# Autodesk Inventor assembly: Final Assembly
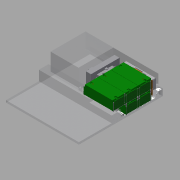
[picture p0: Inventor's stored thumbnail of the model, 180x180]
Saved by Autodesk Inventor 2017 (Build 210142000, 142)
## iProperties
Created: 2022-08-16
Part Number: Final Assembly
Document SubType Name: Assembly
Designer: JTS
Author: JTS
## Documents named in this file (18)
- C:\Users\Windermac\Desktop\MASTER Honda Insight G1 IMA Bay\02 Final Assembly (Tray Mated).iam
- C:\Users\Windermac\Desktop\MASTER Honda Insight G1 IMA Bay\LiBCM003 - Battery Tray\47 Ah FoMoCo Aluminum Tray.ipt
- C:\Users\Windermac\Desktop\MASTER Honda Insight G1 IMA Bay\OEM Parts\Junction Board.ipt
- C:\Users\Windermac\Desktop\MASTER Honda Insight G1 IMA Bay\OEM Parts\MCM.ipt
- C:\Users\Windermac\Desktop\MASTER Honda Insight G1 IMA Bay\Battery Modules\47Ah-FoMoCo.ipt
- C:\Users\Windermac\Desktop\MASTER Honda Insight G1 IMA Bay\LiBCM004 - Battery Rail\Bracket - 5th Module 8982K875.ipt
- C:\Users\Windermac\Desktop\MASTER Honda Insight G1 IMA Bay\Nuts & Bolts\Ring Terminal.ipt
- C:\Users\Windermac\Desktop\MASTER Honda Insight G1 IMA Bay\Final Assembly\AIP\Cable and Harness\Final Assembly.Harness2.iam
- C:\Users\Windermac\Desktop\MASTER Honda Insight G1 IMA Bay\LiBCM PCB\LiBCM Safety Cover - RevC.ipt
- C:\Users\Windermac\Desktop\MASTER Honda Insight G1 IMA Bay\LiBCM PCB\PCB.ipt
- C:\Users\Windermac\Desktop\MASTER Honda Insight G1 IMA Bay\OEM Parts\IMA Bay - Battery Enclosure Interface.ipt
- C:\Users\Windermac\Desktop\MASTER Honda Insight G1 IMA Bay\Nuts & Bolts\Battery Bolt.iam
- C:\Users\Windermac\Desktop\MASTER Honda Insight G1 IMA Bay\Nuts & Bolts\Threaded Standoff.ipt
- C:\Users\Windermac\Desktop\MASTER Honda Insight G1 IMA Bay\Nuts & Bolts\Battery Bolt - Split Washer.iam
- C:\Users\Windermac\Desktop\MASTER Honda Insight G1 IMA Bay\Nuts & Bolts\Washer 0.250in 92141A029.ipt
- C:\Users\Windermac\Desktop\MASTER Honda Insight G1 IMA Bay\Nuts & Bolts\Nut - Hex - 0.250in-20 91845A029.ipt
- C:\Users\Windermac\Desktop\MASTER Honda Insight G1 IMA Bay\Nuts & Bolts\Washer - Split - 92146A029.ipt
- C:\Users\Windermac\Desktop\MASTER Honda Insight G1 IMA Bay\Nuts & Bolts\Top Spacer.ipt
## Components (63 placed, 17 different names)
1. IMA Bay - Battery Enclosure Interface:1 — Insert:56, Mate:2, Mate:3, Mate:4
2. Junction Board:1 — Insert:11, Insert:12
3. MCM:1 — Insert:9, Insert:10
4. Harness2 [sub-assembly]
5. Washer 0.250in 92141A029:3 — Insert:124
6. Nut - Hex - 0.250in-20 91845A029:5
7. Top Spacer:1 — Insert:125, Insert:126
8. 47 Ah FoMoCo Aluminum Tray:1 — Insert:9, Insert:10, Insert:11, Insert:12, Insert:56, Mate:2, Insert:97, Insert:98, Insert:99, Insert:100, Insert:101, Insert:102, Insert:103, Insert:104, Insert:105, Insert:106, Insert:107, Insert:108, Insert:124
9. LiBCM Safety Cover - RevC:1 — Insert:55, Mate:1, Mate:3, Flush:1, Mate:4
10. PCB:1 — Insert:55, Mate:1
11. Threaded Standoff:1 — Insert:65
12. Threaded Standoff:2 — Insert:70
13. Threaded Standoff:3 — Insert:71
14. Threaded Standoff:4 — Insert:72, Insert:114
15. Threaded Standoff:5 — Insert:69, Insert:113
16. Threaded Standoff:6 — Insert:68, Insert:110
17. Threaded Standoff:7 — Insert:67
18. Threaded Standoff:8 — Insert:66, Insert:109
19. Battery Bolt:1 [sub-assembly] — Insert:102
20. Battery Bolt:2 [sub-assembly] — Insert:101
21. Battery Bolt:3 [sub-assembly] — Insert:99
22. Battery Bolt:4 [sub-assembly] — Insert:98
23. Battery Bolt:5 [sub-assembly] — Insert:100
24. Battery Bolt:6 [sub-assembly] — Insert:104
25. Battery Bolt:7 [sub-assembly] — Insert:103
26. Battery Bolt:8 [sub-assembly] — Insert:97
27. 47Ah-FoMoCo:1 — Insert:41, Insert:43, Tangent:1, Tangent:7, Insert:65, Insert:66, Insert:71, Insert:72, Insert:107, Insert:108
28. 47Ah-FoMoCo:2 — Insert:42, Insert:44, Tangent:3, Tangent:13, Insert:67, Insert:68, Insert:69, Insert:70, Insert:105, Insert:106
29. Bracket - 5th Module 8982K875:1 — Insert:109, Insert:110, Insert:111, Insert:112, Insert:120, Insert:121, Insert:122
30. Bracket - 5th Module 8982K875:2 — Insert:113, Insert:114, Insert:115, Insert:116, Insert:117, Insert:118, Insert:119
31. Battery Bolt:9 [sub-assembly] — Insert:115
32. Battery Bolt:10 [sub-assembly] — Insert:116
33. Washer 0.250in 92141A029:1 — Insert:91, Insert:112
34. Washer 0.250in 92141A029:2 — Insert:92, Insert:111
35. Nut - Hex - 0.250in-20 91845A029:1 — Insert:91
36. Nut - Hex - 0.250in-20 91845A029:2 — Insert:92
37. Washer - Split - 92146A029:1 — Insert:93, Insert:95
38. Washer - Split - 92146A029:2 — Insert:94, Insert:96
39. Nut - Hex - 0.250in-20 91845A029:3 — Insert:96
40. Nut - Hex - 0.250in-20 91845A029:4 — Insert:95
41. Battery Bolt - Split Washer:1 [sub-assembly] — Insert:77
42. Battery Bolt - Split Washer:2 [sub-assembly] — Insert:78
43. Battery Bolt - Split Washer:3 [sub-assembly] — Insert:79
44. Battery Bolt - Split Washer:4 [sub-assembly] — Insert:80
45. Battery Bolt - Split Washer:5 [sub-assembly] — Insert:84
46. Battery Bolt - Split Washer:6 [sub-assembly] — Insert:83
47. Battery Bolt - Split Washer:7 [sub-assembly] — Insert:82
48. Battery Bolt - Split Washer:8 [sub-assembly] — Insert:81
49. Battery Bolt - Split Washer:9 [sub-assembly] — Insert:126
50. Battery Bolt - Split Washer:10 [sub-assembly] — Insert:85
51. 47Ah-FoMoCo:3 — Insert:37, Insert:40, Tangent:9, Tangent:12, Flush:1, Insert:79, Insert:80, Insert:81, Insert:82, Insert:121, Insert:122
52. 47Ah-FoMoCo:4 — Insert:36, Insert:39, Tangent:14, Tangent:15, Insert:77, Insert:78, Insert:83, Insert:84, Insert:119, Insert:120
53. 47Ah-FoMoCo:5 — Insert:35, Insert:38, Tangent:16, Tangent:17, Insert:85, Insert:93, Insert:94, Insert:117, Insert:118, Insert:125
54. Ring Terminal:1 — Insert:35, Tangent:16
55. Ring Terminal:2 — Insert:36, Tangent:15
56. Ring Terminal:3 — Insert:37, Tangent:9
57. Ring Terminal:4 — Insert:38, Tangent:17
58. Ring Terminal:5 — Insert:39, Tangent:14
59. Ring Terminal:6 — Insert:40, Tangent:12
60. Ring Terminal:7 — Insert:41, Tangent:1
61. Ring Terminal:8 — Insert:42, Tangent:13
62. Ring Terminal:9 — Insert:43, Tangent:7
63. Ring Terminal:10 — Insert:44, Tangent:3
## Relationships (84: Insert 69, Tangent 10, Mate 4, Flush 1)
- Insert:9: MCM:1 ↔ 47 Ah FoMoCo Aluminum Tray:1
- Insert:10: MCM:1 ↔ 47 Ah FoMoCo Aluminum Tray:1
- Insert:11: Junction Board:1 ↔ 47 Ah FoMoCo Aluminum Tray:1
- Insert:12: Junction Board:1 ↔ 47 Ah FoMoCo Aluminum Tray:1
- Insert:35: 47Ah-FoMoCo:5 ↔ Ring Terminal:1
- Insert:36: 47Ah-FoMoCo:4 ↔ Ring Terminal:2
- Insert:37: 47Ah-FoMoCo:3 ↔ Ring Terminal:3
- Insert:38: 47Ah-FoMoCo:5 ↔ Ring Terminal:4
- Insert:39: 47Ah-FoMoCo:4 ↔ Ring Terminal:5
- Insert:40: 47Ah-FoMoCo:3 ↔ Ring Terminal:6
- Insert:41: 47Ah-FoMoCo:1 ↔ Ring Terminal:7
- Insert:42: 47Ah-FoMoCo:2 ↔ Ring Terminal:8
- Insert:43: 47Ah-FoMoCo:1 ↔ Ring Terminal:9
- Insert:44: 47Ah-FoMoCo:2 ↔ Ring Terminal:10
- Tangent:1 (2 mm): 47Ah-FoMoCo:1 ↔ Ring Terminal:7
- Tangent:3 (4 mm): 47Ah-FoMoCo:2 ↔ Ring Terminal:10
- Tangent:7 (6 mm): 47Ah-FoMoCo:1 ↔ Ring Terminal:9
- Tangent:9 (2 mm): 47Ah-FoMoCo:3 ↔ Ring Terminal:3
- Tangent:12 (2 mm): 47Ah-FoMoCo:3 ↔ Ring Terminal:6
- Tangent:13 (2 mm): 47Ah-FoMoCo:2 ↔ Ring Terminal:8
- Tangent:14 (2 mm): 47Ah-FoMoCo:4 ↔ Ring Terminal:5
- Tangent:15 (2 mm): 47Ah-FoMoCo:4 ↔ Ring Terminal:2
- Tangent:16 (2 mm): 47Ah-FoMoCo:5 ↔ Ring Terminal:1
- Tangent:17 (2 mm): 47Ah-FoMoCo:5 ↔ Ring Terminal:4
- Insert:55 (37 mm): LiBCM Safety Cover - RevC:1 ↔ PCB:1
- Mate:1: LiBCM Safety Cover - RevC:1 ↔ PCB:1
- Insert:56: IMA Bay - Battery Enclosure Interface:1 ↔ 47 Ah FoMoCo Aluminum Tray:1
- Mate:2: IMA Bay - Battery Enclosure Interface:1 ↔ 47 Ah FoMoCo Aluminum Tray:1
- Mate:3 (5 mm): IMA Bay - Battery Enclosure Interface:1 ↔ LiBCM Safety Cover - RevC:1
- Flush:1 (45 mm): LiBCM Safety Cover - RevC:1 ↔ 47Ah-FoMoCo:3
- Mate:4 (31.5 mm): IMA Bay - Battery Enclosure Interface:1 ↔ LiBCM Safety Cover - RevC:1
- Insert:65: Threaded Standoff:1 ↔ 47Ah-FoMoCo:1
- Insert:66: Threaded Standoff:8 ↔ 47Ah-FoMoCo:1
- Insert:67: Threaded Standoff:7 ↔ 47Ah-FoMoCo:2
- Insert:68: Threaded Standoff:6 ↔ 47Ah-FoMoCo:2
- Insert:69: Threaded Standoff:5 ↔ 47Ah-FoMoCo:2
- Insert:70: Threaded Standoff:2 ↔ 47Ah-FoMoCo:2
- Insert:71: Threaded Standoff:3 ↔ 47Ah-FoMoCo:1
- Insert:72: Threaded Standoff:4 ↔ 47Ah-FoMoCo:1
- Insert:77: Battery Bolt - Split Washer:1 ↔ 47Ah-FoMoCo:4
- Insert:78: Battery Bolt - Split Washer:2 ↔ 47Ah-FoMoCo:4
- Insert:79: Battery Bolt - Split Washer:3 ↔ 47Ah-FoMoCo:3
- Insert:80: Battery Bolt - Split Washer:4 ↔ 47Ah-FoMoCo:3
- Insert:81: Battery Bolt - Split Washer:8 ↔ 47Ah-FoMoCo:3
- Insert:82: Battery Bolt - Split Washer:7 ↔ 47Ah-FoMoCo:3
- Insert:83: Battery Bolt - Split Washer:6 ↔ 47Ah-FoMoCo:4
- Insert:84: Battery Bolt - Split Washer:5 ↔ 47Ah-FoMoCo:4
- Insert:85: Battery Bolt - Split Washer:10 ↔ 47Ah-FoMoCo:5
- Insert:91: Washer 0.250in 92141A029:1 ↔ Nut - Hex - 0.250in-20 91845A029:1
- Insert:92: Washer 0.250in 92141A029:2 ↔ Nut - Hex - 0.250in-20 91845A029:2
- Insert:93: Washer - Split - 92146A029:1 ↔ 47Ah-FoMoCo:5
- Insert:94: Washer - Split - 92146A029:2 ↔ 47Ah-FoMoCo:5
- Insert:95: Washer - Split - 92146A029:1 ↔ Nut - Hex - 0.250in-20 91845A029:4
- Insert:96: Washer - Split - 92146A029:2 ↔ Nut - Hex - 0.250in-20 91845A029:3
- Insert:97: 47 Ah FoMoCo Aluminum Tray:1 ↔ Battery Bolt:8
- Insert:98: 47 Ah FoMoCo Aluminum Tray:1 ↔ Battery Bolt:4
- Insert:99: 47 Ah FoMoCo Aluminum Tray:1 ↔ Battery Bolt:3
- Insert:100: 47 Ah FoMoCo Aluminum Tray:1 ↔ Battery Bolt:5
- Insert:101: 47 Ah FoMoCo Aluminum Tray:1 ↔ Battery Bolt:2
- Insert:102: 47 Ah FoMoCo Aluminum Tray:1 ↔ Battery Bolt:1
- Insert:103: 47 Ah FoMoCo Aluminum Tray:1 ↔ Battery Bolt:7
- Insert:104: 47 Ah FoMoCo Aluminum Tray:1 ↔ Battery Bolt:6
- Insert:105: 47 Ah FoMoCo Aluminum Tray:1 ↔ 47Ah-FoMoCo:2
- Insert:106: 47 Ah FoMoCo Aluminum Tray:1 ↔ 47Ah-FoMoCo:2
- Insert:107: 47 Ah FoMoCo Aluminum Tray:1 ↔ 47Ah-FoMoCo:1
- Insert:108: 47 Ah FoMoCo Aluminum Tray:1 ↔ 47Ah-FoMoCo:1
- Insert:109: Threaded Standoff:8 ↔ Bracket - 5th Module 8982K875:1
- Insert:110: Threaded Standoff:6 ↔ Bracket - 5th Module 8982K875:1
- Insert:111: Bracket - 5th Module 8982K875:1 ↔ Washer 0.250in 92141A029:2
- Insert:112: Bracket - 5th Module 8982K875:1 ↔ Washer 0.250in 92141A029:1
- Insert:113: Threaded Standoff:5 ↔ Bracket - 5th Module 8982K875:2
- Insert:114: Threaded Standoff:4 ↔ Bracket - 5th Module 8982K875:2
- Insert:115: Bracket - 5th Module 8982K875:2 ↔ Battery Bolt:9
- Insert:116: Bracket - 5th Module 8982K875:2 ↔ Battery Bolt:10
- Insert:117: Bracket - 5th Module 8982K875:2 ↔ 47Ah-FoMoCo:5
- Insert:118: Bracket - 5th Module 8982K875:2 ↔ 47Ah-FoMoCo:5
- Insert:119: Bracket - 5th Module 8982K875:2 ↔ 47Ah-FoMoCo:4
- Insert:120: Bracket - 5th Module 8982K875:1 ↔ 47Ah-FoMoCo:4
- Insert:121: Bracket - 5th Module 8982K875:1 ↔ 47Ah-FoMoCo:3
- Insert:122: Bracket - 5th Module 8982K875:1 ↔ 47Ah-FoMoCo:3
- [Insert]: Washer 0.250in 92141A029:3 ↔ Nut - Hex - 0.250in-20 91845A029:5
- Insert:124: Washer 0.250in 92141A029:3 ↔ 47 Ah FoMoCo Aluminum Tray:1
- Insert:125: Top Spacer:1 ↔ 47Ah-FoMoCo:5
- Insert:126: Top Spacer:1 ↔ Battery Bolt - Split Washer:9
## Named parameters: d147_d115 = 0 mm
